# Autodesk Inventor assembly: Servo_aseem
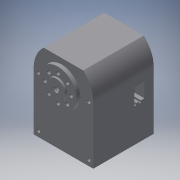
[picture p0: Inventor's stored thumbnail of the model, 180x180]
Saved by Autodesk Inventor 2016 (Build 200138000, 138)
## iProperties
Created: 2015-09-14
Part Number: Servo_aseem
Material: 一般
Document SubType Name: Assembly
Designer: daisuke
Mass: 41.0048 g
Surface Area: 101.286 cm^2
Volume: 43.0399 cm^3
Density: 0.952716 g/cm^3
Author: daisuke
## Documents named in this file (3)
- C:\Users\宏太\Documents\GitHub\Tomato2016\Servo.iam
- C:\Users\宏太\Documents\GitHub\Tomato2016\FreeHorn.ipt
- C:\Users\宏太\Documents\GitHub\Tomato2016\Servo.ipt
## Components (2 placed, 2 different names)
1. FreeHorn:1 — 挿入:1
2. Servo:1 — 挿入:1
## Relationships (1: Insert 1)
- 挿入:1 [Insert]: FreeHorn:1 ↔ Servo:1
